# Autodesk Inventor assembly: Assembly_Insert_Kinematic_Mirrormount_45_base-Kopie
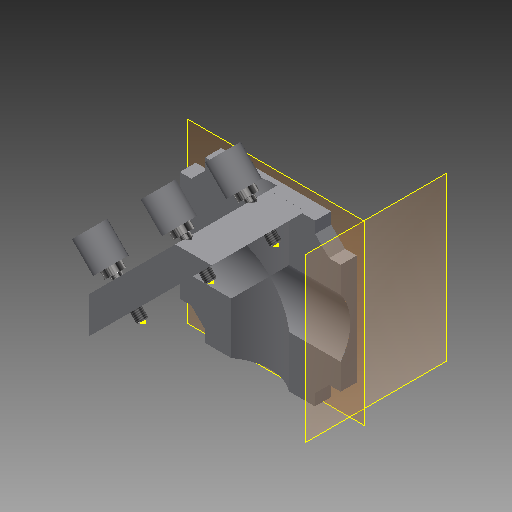
[picture p0: Inventor's stored thumbnail of the model, 512x512]
Saved by Autodesk Inventor 2019 (Build 230136000, 136)
## iProperties
Created: 2020-12-03
Part Number: Assembly_Insert_Kinematic_Mirrormount_45_base-Kopie
Document SubType Name: Assembly
Designer: wanghaoran
Author: wanghaoran
## Documents named in this file (5)
- C:\Users\marsikovabarbora\Dropbox\UC2\02_CAD\INVENTOR\uc2_v3\Assembly_Insert_Kinematic_Mirrormount_45_base-Kopie.iam
- C:\Users\marsikovabarbora\Dropbox\UC2\02_CAD\INVENTOR\uc2_v3\20_Cube_Insert_Kinematic_Mirrormount_45_base_part1.ipt
- C:\Users\marsikovabarbora\Dropbox\UC2\02_CAD\INVENTOR\uc2_v3\20_Cube_Insert_Kinematic_Mirrormount_45_base_part2.ipt
- C:\Users\marsikovabarbora\Dropbox\UC2\02_CAD\INVENTOR\uc2_v3\30_Adapter_M3_nut.ipt
- C:\Users\marsikovabarbora\Dropbox\UC2\02_CAD\INVENTOR\uc2_v3\openSIMv3\BAK\DIN 912 - M3 x 0,5 x 12 x 10,75.ipt
## Components (8 placed, 4 different names)
1. 20_Cube_Insert_Kinematic_Mirrormount_45_base_part1:1 — Mate:1, Mate:2, Mate:3
2. 20_Cube_Insert_Kinematic_Mirrormount_45_base_part2:1 — Mate:1, Mate:2, Mate:3, Mate:4, Mate:5, Mate:6, Mate:7, Mate:8, Mate:9, Mate:10, Mate:11, Mate:12, Mate:13, Mate:14, Flush:1
3. 30_Adapter_M3_nut:1 — Mate:4, Mate:7
4. 30_Adapter_M3_nut:2 — Mate:5, Mate:9
5. 30_Adapter_M3_nut:3 — Mate:6, Mate:8
6. DIN 912 - ersetzt durch DIN EN ISO 4762 M3 x 12:1 — Mate:10, Mate:11
7. DIN 912 - ersetzt durch DIN EN ISO 4762 M3 x 12:2 — Mate:12, Mate:14
8. DIN 912 - ersetzt durch DIN EN ISO 4762 M3 x 12:3 — Mate:13, Flush:1
## Relationships (15: Mate 14, Flush 1)
- Mate:1: 20_Cube_Insert_Kinematic_Mirrormount_45_base_part1:1 ↔ 20_Cube_Insert_Kinematic_Mirrormount_45_base_part2:1
- Mate:2: 20_Cube_Insert_Kinematic_Mirrormount_45_base_part1:1 ↔ 20_Cube_Insert_Kinematic_Mirrormount_45_base_part2:1
- Mate:3: 20_Cube_Insert_Kinematic_Mirrormount_45_base_part1:1 ↔ 20_Cube_Insert_Kinematic_Mirrormount_45_base_part2:1
- Mate:4: 20_Cube_Insert_Kinematic_Mirrormount_45_base_part2:1 ↔ 30_Adapter_M3_nut:1
- Mate:5: 20_Cube_Insert_Kinematic_Mirrormount_45_base_part2:1 ↔ 30_Adapter_M3_nut:2
- Mate:6: 20_Cube_Insert_Kinematic_Mirrormount_45_base_part2:1 ↔ 30_Adapter_M3_nut:3
- Mate:7 (3 mm): 20_Cube_Insert_Kinematic_Mirrormount_45_base_part2:1 ↔ 30_Adapter_M3_nut:1
- Mate:8 (3 mm): 20_Cube_Insert_Kinematic_Mirrormount_45_base_part2:1 ↔ 30_Adapter_M3_nut:3
- Mate:9 (3 mm): 20_Cube_Insert_Kinematic_Mirrormount_45_base_part2:1 ↔ 30_Adapter_M3_nut:2
- Mate:10: 20_Cube_Insert_Kinematic_Mirrormount_45_base_part2:1 ↔ DIN 912 - ersetzt durch DIN EN ISO 4762 M3 x 12:1
- Mate:11 (3 mm): 20_Cube_Insert_Kinematic_Mirrormount_45_base_part2:1 ↔ DIN 912 - ersetzt durch DIN EN ISO 4762 M3 x 12:1
- Mate:12: 20_Cube_Insert_Kinematic_Mirrormount_45_base_part2:1 ↔ DIN 912 - ersetzt durch DIN EN ISO 4762 M3 x 12:2
- Mate:13: 20_Cube_Insert_Kinematic_Mirrormount_45_base_part2:1 ↔ DIN 912 - ersetzt durch DIN EN ISO 4762 M3 x 12:3
- Mate:14 (3 mm): 20_Cube_Insert_Kinematic_Mirrormount_45_base_part2:1 ↔ DIN 912 - ersetzt durch DIN EN ISO 4762 M3 x 12:2
- Flush:1 (-3 mm): 20_Cube_Insert_Kinematic_Mirrormount_45_base_part2:1 ↔ DIN 912 - ersetzt durch DIN EN ISO 4762 M3 x 12:3
